# Autodesk Inventor assembly: Assembly1
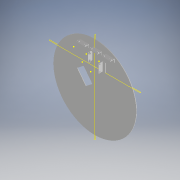
[picture p0: Inventor's stored thumbnail of the model, 180x180]
Saved by Autodesk Inventor 2020 (Build 240168000, 168)
## iProperties
Created: 2020-07-11
Part Number: Assembly1
Document SubType Name: Assembly
Designer: Sičaja
Author: Sičaja
## Documents named in this file (3)
- C:\Users\Sicaja\Documents\Draws_Inventor\Robocup_robot\Assembly1.iam
- C:\Users\Sicaja\Documents\Draws_Inventor\Robocup_robot\GonjaKonstrukcija_v.1.0.ipt
- C:\Users\Sicaja\Documents\Draws_Inventor\Robocup_robot\5DržačaLidara.ipt
## Components (2 placed, 2 different names)
1. GonjaKonstrukcija_v.1.0:1 — Mate:1, Flush:1, Mate:2, Mate:3
2. 5DržačaLidara:1 — Mate:1, Mate:4, Mate:5
## Relationships (6: Mate 5, Flush 1)
- Mate:1: GonjaKonstrukcija_v.1.0:1 ↔ 5DržačaLidara:1
- Flush:1 (-1 mm): GonjaKonstrukcija_v.1.0:1
- Mate:2: GonjaKonstrukcija_v.1.0:1
- Mate:3: GonjaKonstrukcija_v.1.0:1
- Mate:4 (-3 mm): 5DržačaLidara:1
- Mate:5: 5DržačaLidara:1
